# Autodesk Inventor assembly: 1Ufullsystem
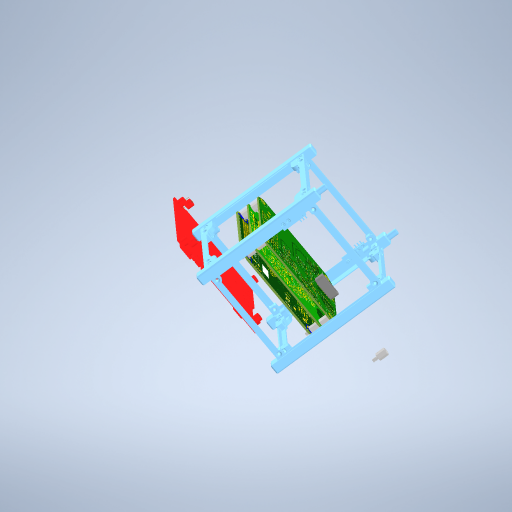
[picture p0: Inventor's stored thumbnail of the model, 512x512]
Saved by Autodesk Inventor 2024 (Build 280153000, 153)
## iProperties
Created: 2023-04-12
Part Number: 1Ufullsystem
Document SubType Name: Assembly
Designer: User
Author: User
## Documents named in this file (7)
- C:\Users\User\Documents\1UFrame\1Ufullsystem.iam
- C:\Users\User\Documents\1UFrame\ISISpace\ISIS CubeSat STS PC104 Skeleton.iam
- C:\Users\User\Documents\1UFrame\PCB_LT_ICR.iam
- C:\Users\User\Documents\1UFrame\PCB_LT_RX-TX.iam
- C:\Users\User\Documents\1UFrame\PCB_LIHU.iam
- C:\Users\User\Documents\1UFrame\PC104_EM-113 Assembly.iam
- C:\Users\User\Downloads\93655A419_Male-Female Threaded Hex Standoff\93655A419_Male-Female Threaded Hex Standoff.ipt
## Components (14 placed, 6 different names)
1. ISIS CubeSat STS PC104 Skeleton:1 [sub-assembly]
2. PCB_LT_ICR:1 [sub-assembly] — Mate:82, Mate:83, Mate:86, Mate:87, Mate:90, Mate:91, Mate:93, Mate:94
3. PCB_LT_RX-TX:1 [sub-assembly] — Mate:80, Mate:81, Mate:84, Mate:85, Mate:88, Mate:89, Mate:92, Mate:97, Mate:101, Mate:105, Mate:108
4. PCB_LIHU:2 [sub-assembly] — Mate:95, Mate:99, Mate:100, Mate:103, Mate:104, Mate:106, Mate:107
5. PC104_EM-113 Assembly:1 [sub-assembly]
6. 93655A419_Male-Female Threaded Hex Standoff:1 — Mate:88, Mate:89, Mate:90, Mate:91
7. 93655A419_Male-Female Threaded Hex Standoff:2 — Mate:84, Mate:85, Mate:86, Mate:87, Mate:98
8. 93655A419_Male-Female Threaded Hex Standoff:3 — Mate:92, Mate:93, Mate:94
9. 93655A419_Male-Female Threaded Hex Standoff:4 — Mate:80, Mate:81, Mate:82, Mate:83, Mate:102
10. 93655A419_Male-Female Threaded Hex Standoff:5 — Mate:95, Mate:97, Mate:98
11. 93655A419_Male-Female Threaded Hex Standoff:6 — Mate:99, Mate:100, Mate:101, Mate:102
12. 93655A419_Male-Female Threaded Hex Standoff:7 — Mate:103, Mate:104, Mate:105
13. 93655A419_Male-Female Threaded Hex Standoff:8 — Mate:106, Mate:107, Mate:108
14. 93655A419_Male-Female Threaded Hex Standoff:9
## Relationships (28: Mate 28)
- Mate:80: PCB_LT_RX-TX:1 ↔ 93655A419_Male-Female Threaded Hex Standoff:4
- Mate:81: PCB_LT_RX-TX:1 ↔ 93655A419_Male-Female Threaded Hex Standoff:4
- Mate:82: PCB_LT_ICR:1 ↔ 93655A419_Male-Female Threaded Hex Standoff:4
- Mate:83: PCB_LT_ICR:1 ↔ 93655A419_Male-Female Threaded Hex Standoff:4
- Mate:84: PCB_LT_RX-TX:1 ↔ 93655A419_Male-Female Threaded Hex Standoff:2
- Mate:85: PCB_LT_RX-TX:1 ↔ 93655A419_Male-Female Threaded Hex Standoff:2
- Mate:86: PCB_LT_ICR:1 ↔ 93655A419_Male-Female Threaded Hex Standoff:2
- Mate:87: PCB_LT_ICR:1 ↔ 93655A419_Male-Female Threaded Hex Standoff:2
- Mate:88: PCB_LT_RX-TX:1 ↔ 93655A419_Male-Female Threaded Hex Standoff:1
- Mate:89: PCB_LT_RX-TX:1 ↔ 93655A419_Male-Female Threaded Hex Standoff:1
- Mate:90: PCB_LT_ICR:1 ↔ 93655A419_Male-Female Threaded Hex Standoff:1
- Mate:91: PCB_LT_ICR:1 ↔ 93655A419_Male-Female Threaded Hex Standoff:1
- Mate:92: PCB_LT_RX-TX:1 ↔ 93655A419_Male-Female Threaded Hex Standoff:3
- Mate:93: PCB_LT_ICR:1 ↔ 93655A419_Male-Female Threaded Hex Standoff:3
- Mate:94: PCB_LT_ICR:1 ↔ 93655A419_Male-Female Threaded Hex Standoff:3
- Mate:95: PCB_LIHU:2 ↔ 93655A419_Male-Female Threaded Hex Standoff:5
- Mate:97: PCB_LT_RX-TX:1 ↔ 93655A419_Male-Female Threaded Hex Standoff:5
- Mate:98: 93655A419_Male-Female Threaded Hex Standoff:2 ↔ 93655A419_Male-Female Threaded Hex Standoff:5
- Mate:99: PCB_LIHU:2 ↔ 93655A419_Male-Female Threaded Hex Standoff:6
- Mate:100: PCB_LIHU:2 ↔ 93655A419_Male-Female Threaded Hex Standoff:6
- Mate:101: PCB_LT_RX-TX:1 ↔ 93655A419_Male-Female Threaded Hex Standoff:6
- Mate:102: 93655A419_Male-Female Threaded Hex Standoff:4 ↔ 93655A419_Male-Female Threaded Hex Standoff:6
- Mate:103: PCB_LIHU:2 ↔ 93655A419_Male-Female Threaded Hex Standoff:7
- Mate:104: PCB_LIHU:2 ↔ 93655A419_Male-Female Threaded Hex Standoff:7
- Mate:105: PCB_LT_RX-TX:1 ↔ 93655A419_Male-Female Threaded Hex Standoff:7
- Mate:106: PCB_LIHU:2 ↔ 93655A419_Male-Female Threaded Hex Standoff:8
- Mate:107: PCB_LIHU:2 ↔ 93655A419_Male-Female Threaded Hex Standoff:8
- Mate:108: PCB_LT_RX-TX:1 ↔ 93655A419_Male-Female Threaded Hex Standoff:8
